# Autodesk Inventor assembly: Bot 1
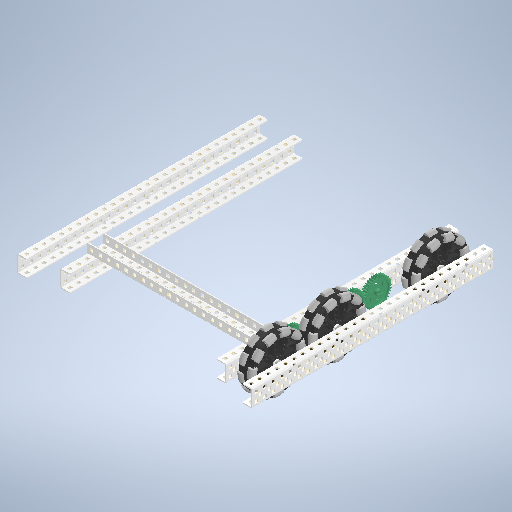
[picture p0: Inventor's stored thumbnail of the model, 512x512]
Saved by Autodesk Inventor 2025.2 (Build 292293000, 293)
## iProperties
Created: 2025-03-17
Part Number: Bot 1
Document SubType Name: Assembly
Designer: Jahan
Author: Jahan
## Documents named in this file (16)
- C:\1629X-7700R-Worlds-Bot\Bot 1\Bot 1.iam
- C:\1629X-7700R-Worlds-Bot\VEX-CAD-Inventor-1.4.2\Structure\C Channel\Aluminum 1x2x1\Alu C 1x2x1x27.ipt
- C:\1629X-7700R-Worlds-Bot\VEX-CAD-Inventor-1.4.2\Structure\C Channel\Aluminum 1x2x1\Alu C 1x2x1x19.ipt
- C:\1629X-7700R-Worlds-Bot\VEX-CAD-Inventor-1.4.2\Structure\C Channel\Aluminum 1x2x1\Alu C 1x2x1x28.ipt
- C:\1629X-7700R-Worlds-Bot\VEX-CAD-Inventor-1.4.2\Motion\Gears\HS Gear.iam
- C:\1629X-7700R-Worlds-Bot\VEX-CAD-Inventor-1.4.2\Motion\Wheels\Omni Wheel\3.25 Omni AS, No Insert.iam
- C:\1629X-7700R-Worlds-Bot\VEX-CAD-Inventor-1.4.2\Motion\Wheels\Omni Wheel.iam
- C:\1629X-7700R-Worlds-Bot\VEX-CAD-Inventor-1.4.2\Motion\Gears\HS Gear\HS 48T Gear, Circle.iam
- C:\1629X-7700R-Worlds-Bot\VEX-CAD-Inventor-1.4.2\Structure\Standoff.ipt
- C:\1629X-7700R-Worlds-Bot\VEX-CAD-Inventor-1.4.2\Structure\Standoff\Standoff .50.ipt
- C:\1629X-7700R-Worlds-Bot\VEX-CAD-Inventor-1.4.2\Motion\Spacers\Washer Teflon.ipt
- C:\1629X-7700R-Worlds-Bot\VEX-CAD-Inventor-1.4.2\Motion\Spacers\Spacer Nylon .375 OD\NSpacer .375 OD x .125.ipt
- C:\1629X-7700R-Worlds-Bot\VEX-CAD-Inventor-1.4.2\Motion\Spacers\Spacer Nylon .375 OD.ipt
- C:\1629X-7700R-Worlds-Bot\VEX-CAD-Inventor-1.4.2\Motion\Spacers\Washer Teflon\TWasher .375 OD x .06250.ipt
- C:\1629X-7700R-Worlds-Bot\VEX-CAD-Inventor-1.4.2\Structure\Hardware\alu_nylock.ipt
- C:\1629X-7700R-Worlds-Bot\VEX-CAD-Inventor-1.4.2\Motion\Gears\LS 36T Gear.ipt
## Components (27 placed, 10 different names)
1. Alu C 1x2x1x19:1 — Insert:1, Insert:2, Insert:3, Insert:4
2. Alu C 1x2x1x27:1 — Insert:3, Insert:4, Insert:19, Insert:32, Insert:33
3. Alu C 1x2x1x27:2 — Insert:1, Insert:2, Insert:5, Insert:6
4. Alu C 1x2x1x27:3 — Insert:5, Insert:6, Insert:7, Insert:8, Insert:9, Insert:10
5. Alu C 1x2x1x28:1 — Insert:7, Insert:8
6. Alu C 1x2x1x28:2 — Insert:9, Insert:10, Insert:25, Insert:31, Insert:39
7. LS 36T Gear:1 — Insert:19
8. HS 48T Gear, Circle:3 [sub-assembly]
9. 3.25 Omni AS, No Insert:4 [sub-assembly]
10. NSpacer .375 OD x .125:2
11. TWasher .375 OD x .06250:2 — Insert:23
12. alu_nylock:3 — Insert:23, Insert:24
13. Standoff .50:3 — Insert:24, Insert:25
14. HS 48T Gear, Circle:4 [sub-assembly]
15. 3.25 Omni AS, No Insert:5 [sub-assembly]
16. NSpacer .375 OD x .125:3
17. TWasher .375 OD x .06250:3
18. alu_nylock:4
19. Standoff .50:4 — Insert:31
20. LS 36T Gear:2 — Insert:32
21. LS 36T Gear:3 — Insert:33
22. HS 48T Gear, Circle:5 [sub-assembly]
23. 3.25 Omni AS, No Insert:6 [sub-assembly]
24. NSpacer .375 OD x .125:4
25. TWasher .375 OD x .06250:4
26. alu_nylock:5
27. Standoff .50:5 — Insert:39
## Relationships (31: Insert 31)
- Insert:1: Alu C 1x2x1x19:1 ↔ Alu C 1x2x1x27:2
- Insert:2: Alu C 1x2x1x19:1 ↔ Alu C 1x2x1x27:2
- Insert:3: Alu C 1x2x1x19:1 ↔ Alu C 1x2x1x27:1
- Insert:4: Alu C 1x2x1x19:1 ↔ Alu C 1x2x1x27:1
- Insert:5: Alu C 1x2x1x27:2 ↔ Alu C 1x2x1x27:3
- Insert:6: Alu C 1x2x1x27:2 ↔ Alu C 1x2x1x27:3
- Insert:7: Alu C 1x2x1x27:3 ↔ Alu C 1x2x1x28:1
- Insert:8: Alu C 1x2x1x27:3 ↔ Alu C 1x2x1x28:1
- Insert:9: Alu C 1x2x1x27:3 ↔ Alu C 1x2x1x28:2
- Insert:10: Alu C 1x2x1x27:3 ↔ Alu C 1x2x1x28:2
- Insert:19: Alu C 1x2x1x27:1 ↔ LS 36T Gear:1
- [Insert]: HS 48T Gear, Circle:3 ↔ 3.25 Omni AS, No Insert:4
- [Insert]: HS 48T Gear, Circle:3 ↔ NSpacer .375 OD x .125:2
- [Insert]: 3.25 Omni AS, No Insert:4 ↔ TWasher .375 OD x .06250:2
- Insert:23: TWasher .375 OD x .06250:2 ↔ alu_nylock:3
- Insert:24: alu_nylock:3 ↔ Standoff .50:3
- Insert:25: Alu C 1x2x1x28:2 ↔ Standoff .50:3
- [Insert]: HS 48T Gear, Circle:4 ↔ 3.25 Omni AS, No Insert:5
- [Insert]: HS 48T Gear, Circle:4 ↔ NSpacer .375 OD x .125:3
- [Insert]: 3.25 Omni AS, No Insert:5 ↔ TWasher .375 OD x .06250:3
- [Insert]: TWasher .375 OD x .06250:3 ↔ alu_nylock:4
- [Insert]: alu_nylock:4 ↔ Standoff .50:4
- Insert:31: Alu C 1x2x1x28:2 ↔ Standoff .50:4
- Insert:32: Alu C 1x2x1x27:1 ↔ LS 36T Gear:2
- Insert:33: Alu C 1x2x1x27:1 ↔ LS 36T Gear:3
- [Insert]: HS 48T Gear, Circle:5 ↔ 3.25 Omni AS, No Insert:6
- [Insert]: HS 48T Gear, Circle:5 ↔ NSpacer .375 OD x .125:4
- [Insert]: 3.25 Omni AS, No Insert:6 ↔ TWasher .375 OD x .06250:4
- [Insert]: TWasher .375 OD x .06250:4 ↔ alu_nylock:5
- [Insert]: alu_nylock:5 ↔ Standoff .50:5
- Insert:39: Alu C 1x2x1x28:2 ↔ Standoff .50:5
## Named parameters: d122_d116 = 0 mm, d123_d117 = 0 mm, d124_d119 = 0 mm, d129_d122_d116 = 0 mm, d130_d123_d117 = 0 mm, d131_d124_d119 = 0 mm, d132_d126 = 0 mm, d133_d127 = 0 mm, d144_d129_d122_d116 = 0 mm, d145_d130_d123_d117 = 0 mm, d146_d131_d124_d119 = 0 mm, d147_d132_d126 = 0 mm, d148_d133_d127 = 0 mm
